# Autodesk Inventor assembly: Assembly1
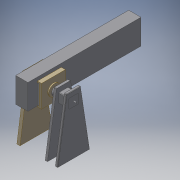
[picture p0: Inventor's stored thumbnail of the model, 180x180]
Saved by Autodesk Inventor 2018 (Build 220112000, 112)
## iProperties
Created: 2018-11-09
Part Number: Assembly1
Document SubType Name: Assembly
Designer: Cameron
Author: Cameron
## Documents named in this file (11)
- C:\Users\Cameron\Documents\Capstone\Gun Design\Assembly1.iam
- C:\Users\Cameron\Documents\Capstone\Gun Design\Nerf Gun.ipt
- C:\Users\Cameron\Documents\Capstone\Gun Design\left gun mount.ipt
- C:\Users\Cameron\Documents\Capstone\Gun Design\Right Gun Mount.ipt
- C:\Users\Cameron\Documents\Capstone\Gun Design\Rotor_Motor.ipt
- C:\Users\Cameron\Documents\Capstone\Gun Design\Motor Mount_2.ipt
- C:\Users\Cameron\Documents\Capstone\Gun Design\Assembly1\AIP\FEA\couu54ps0.fins
- C:\Users\Cameron\Documents\Capstone\Gun Design\Assembly1\AIP\FEA\couu54psw.fsat
- C:\Users\Cameron\Documents\Capstone\Gun Design\Assembly1\AIP\FEA\couu54psw.ftes
- C:\Users\Cameron\Documents\Capstone\Gun Design\Assembly1\AIP\FEA\couu54psw.fwiz
- C:\Users\Cameron\Documents\Capstone\Gun Design\Assembly1\AIP\FEA\couu54puo.fmsh
## Components (5 placed, 5 different names)
1. Nerf Gun:1 — Flush:1, Flush:2, Flush:3, Flush:4, Flush:5, Flush:6, Mate:1, Mate:2, Mate:3, Flush:7
2. left gun mount:1 — Flush:1, Flush:2, Mate:3, Flush:7, Mate:4, Angle:1, Mate:5
3. Right Gun Mount:1 — Flush:3, Flush:4, Flush:5, Flush:6, Mate:1, Mate:2
4. Rotor_Motor:1 — Mate:4, Angle:1, Mate:5, Flush:9, Flush:10
5. Motor Mount_2:1 — Flush:9, Flush:10
## Relationships (15: Flush 9, Mate 5, Angle 1)
- Flush:1: Nerf Gun:1 ↔ left gun mount:1
- Flush:2: Nerf Gun:1 ↔ left gun mount:1
- Flush:3: Nerf Gun:1 ↔ Right Gun Mount:1
- Flush:4: Nerf Gun:1 ↔ Right Gun Mount:1
- Flush:5: Nerf Gun:1 ↔ Right Gun Mount:1
- Flush:6: Nerf Gun:1 ↔ Right Gun Mount:1
- Mate:1: Nerf Gun:1 ↔ Right Gun Mount:1
- Mate:2: Nerf Gun:1 ↔ Right Gun Mount:1
- Mate:3: Nerf Gun:1 ↔ left gun mount:1
- Flush:7: Nerf Gun:1 ↔ left gun mount:1
- Mate:4: left gun mount:1 ↔ Rotor_Motor:1
- Angle:1 (0 deg): left gun mount:1 ↔ Rotor_Motor:1
- Mate:5: left gun mount:1 ↔ Rotor_Motor:1
- Flush:9: Rotor_Motor:1 ↔ Motor Mount_2:1
- Flush:10: Rotor_Motor:1 ↔ Motor Mount_2:1
## Named parameters: sa_0 = -1.33447e-10, sa_1 = -444822, sa_2 = 1.77929e-10
note: some values were not read from the file. Shown as the stored number, unit unknown: "sa_0", "sa_1", "sa_2".
